# Autodesk Inventor assembly: Assembly-payload-part1
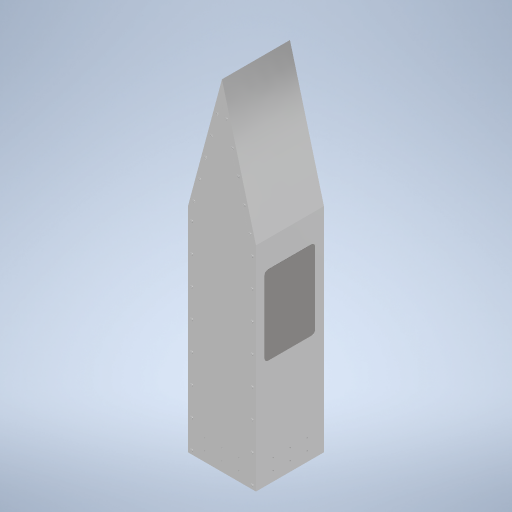
[picture p0: Inventor's stored thumbnail of the model, 512x512]
Saved by Autodesk Inventor 2023 (Build 270158000, 158)
## iProperties
Created: 2023-04-06
Part Number: Assembly-payload-part1
Document SubType Name: Assembly
Designer: ASARe-DAQ-PC
Mass: 73218.4 g
Surface Area: 104206 cm^2
Volume: 27117.9 cm^3
Density: 2.7 g/cm^3
Author: ASARe-DAQ-PC
## Documents named in this file (17)
- C:\Users\310611102\Documents\Inventor\SSR\avionics_2023ver\Payload\Assembly-payload-part1.iam
- C:\Users\310611102\Documents\Inventor\SSR\avionics_2023ver\Payload\Model Shell_part1_up_plate.ipt
- C:\Users\310611102\Documents\Inventor\SSR\avionics_2023ver\Payload\Model Shell_part1_bottom_plate.ipt
- C:\Users\310611102\Documents\Inventor\SSR\avionics_2023ver\Payload\Model Shell_part1_side_plate.ipt
- C:\Users\310611102\Documents\Inventor\SSR\avionics_2023ver\Payload\Model Shell_part1_tip_plate.ipt
- C:\Users\310611102\Documents\Inventor\SSR\avionics_2023ver\Payload\back_board.ipt
- C:\Users\310611102\Documents\Inventor\SSR\avionics_2023ver\Payload\waterproof_door_on_back_board.ipt
- C:\Users\310611102\Documents\Inventor\SSR\avionics_2023ver\Payload\Screw M4 Hex Flat Head 14mm.ipt
- C:\Users\310611102\Documents\Inventor\SSR\avionics_2023ver\Payload\Screw M3 Hex 12mm.ipt
- C:\Users\310611102\Documents\Inventor\SSR\avionics_2023ver\Payload\Screw M4 Hex Flat Head 10mm.ipt
- C:\Users\310611102\Documents\Inventor\SSR\avionics_2023ver\Payload\Screw M3 Hex 8mm.ipt
- C:\Users\310611102\Documents\Inventor\SSR\avionics_2023ver\Payload\Model Shell_part1_side_plate_no_hole.ipt
- C:\Users\310611102\Documents\Inventor\SSR\avionics_2023ver\Payload\Tip_support_1.ipt
- C:\Users\310611102\Documents\Inventor\SSR\avionics_2023ver\Payload\Mirror_shell3.ipt
- C:\Users\310611102\Documents\Inventor\SSR\avionics_2023ver\Payload\acrylic_for_PSI.ipt
- C:\Users\310611102\Documents\Inventor\SSR\avionics_2023ver\Payload\FSI Plate.ipt
- C:\Users\310611102\Documents\Inventor\SSR\avionics_2023ver\Payload\Model Shell - access panel L.ipt
## Components (81 placed, 16 different names)
1. Model Shell_part1_up_plate:1 — Flush:2, Flush:3, Mate:3, Mate:4, Mate:7, Insert:44, Insert:46, Insert:48, Insert:50, Insert:52, Insert:54, Insert:56, Insert:58, Insert:76, Insert:77, Insert:80, Insert:82, Insert:84, Insert:86, Insert:88, Insert:90, Mate:17, Insert:96, Mate:20, Flush:7, Flush:8, Mate:21, Mate:22, Mate:23
2. Model Shell_part1_bottom_plate:1 — Flush:3, Mate:5, Mate:6, Insert:43, Insert:45, Insert:47, Insert:49, Insert:51, Insert:53, Insert:55, Insert:57, Insert:75, Insert:78, Insert:79, Insert:81, Insert:83, Insert:85, Insert:87, Insert:89, Flush:6, Mate:18, Insert:95
3. Model Shell_part1_side_plate:2 — Flush:2, Mate:3, Mate:4, Mate:5, Mate:6, Flush:4, Mate:9, Flush:5, Insert:1, Insert:2, Insert:91, Insert:94, Mate:24, Insert:101, Insert:102
4. Model Shell_part1_tip_plate:1 — Mate:9, Flush:5, Mate:10, Insert:4, Insert:5, Insert:59, Insert:61, Insert:63, Insert:66, Insert:68, Insert:69, Insert:71, Insert:74
5. Model Shell_part1_tip_plate:2 — Mate:7, Flush:4, Mate:10, Insert:3, Insert:6, Insert:60, Insert:62, Insert:64, Insert:65, Insert:67, Insert:70, Insert:72, Insert:73
6. back_board:1 — Insert:1, Insert:2, Mate:14, Mate:15, Mate:16
7. waterproof_door_on_back_board:1 — Mate:14, Mate:15, Mate:16, Insert:31, Insert:32, Insert:33, Insert:34, Insert:35, Insert:36, Insert:37, Insert:38, Insert:39, Insert:40, Insert:41, Insert:42
8. Screw M4 Hex Flat Head 14mm:1 — Insert:3
9. Screw M4 Hex Flat Head 14mm:2 — Insert:4
10. Screw M4 Hex Flat Head 14mm:3 — Insert:5
11. Screw M4 Hex Flat Head 14mm:4 — Insert:6
12. Screw M3 Hex 12mm:1 — Insert:34
13. Screw M3 Hex 12mm:2 — Insert:33
14. Screw M3 Hex 12mm:3 — Insert:32
15. Screw M3 Hex 12mm:4 — Insert:31
16. Screw M3 Hex 12mm:5 — Insert:40
17. Screw M3 Hex 12mm:6 — Insert:41
18. Screw M3 Hex 12mm:7 — Insert:35
19. Screw M3 Hex 12mm:8 — Insert:36
20. Screw M3 Hex 12mm:9 — Insert:37
21. Screw M3 Hex 12mm:10 — Insert:42
22. Screw M3 Hex 12mm:11 — Insert:38
23. Screw M3 Hex 12mm:12 — Insert:39
24. Screw M4 Hex Flat Head 10mm:1 — Insert:66
25. Screw M4 Hex Flat Head 10mm:2 — Insert:65
26. Screw M4 Hex Flat Head 10mm:3 — Insert:64
27. Screw M4 Hex Flat Head 10mm:4 — Insert:63
28. Screw M4 Hex Flat Head 10mm:5 — Insert:62
29. Screw M4 Hex Flat Head 10mm:6 — Insert:61
30. Screw M4 Hex Flat Head 10mm:7 — Insert:60
31. Screw M4 Hex Flat Head 10mm:8 — Insert:59
32. Screw M4 Hex Flat Head 10mm:9 — Insert:58
33. Screw M4 Hex Flat Head 10mm:10 — Insert:57
34. Screw M4 Hex Flat Head 10mm:11 — Insert:56
35. Screw M4 Hex Flat Head 10mm:12 — Insert:55
36. Screw M4 Hex Flat Head 10mm:13 — Insert:54
37. Screw M4 Hex Flat Head 10mm:14 — Insert:53
38. Screw M4 Hex Flat Head 10mm:15 — Insert:52
39. Screw M4 Hex Flat Head 10mm:16 — Insert:51
40. Screw M4 Hex Flat Head 10mm:17 — Insert:50
41. Screw M4 Hex Flat Head 10mm:18 — Insert:49
42. Screw M4 Hex Flat Head 10mm:19 — Insert:48
43. Screw M4 Hex Flat Head 10mm:20 — Insert:47
44. Screw M4 Hex Flat Head 10mm:21 — Insert:46
45. Screw M4 Hex Flat Head 10mm:22 — Insert:45
46. Screw M4 Hex Flat Head 10mm:23 — Insert:43
47. Screw M4 Hex Flat Head 10mm:24 — Insert:44
48. Screw M4 Hex Flat Head 10mm:25 — Insert:90
49. Screw M4 Hex Flat Head 10mm:26 — Insert:89
50. Screw M4 Hex Flat Head 10mm:27 — Insert:87
51. Screw M4 Hex Flat Head 10mm:28 — Insert:88
52. Screw M4 Hex Flat Head 10mm:29 — Insert:85
53. Screw M4 Hex Flat Head 10mm:30 — Insert:86
54. Screw M4 Hex Flat Head 10mm:31 — Insert:83
55. Screw M4 Hex Flat Head 10mm:32 — Insert:84
56. Screw M4 Hex Flat Head 10mm:33 — Insert:81
57. Screw M4 Hex Flat Head 10mm:34 — Insert:82
58. Screw M4 Hex Flat Head 10mm:35 — Insert:79
59. Screw M4 Hex Flat Head 10mm:36 — Insert:80
60. Screw M4 Hex Flat Head 10mm:37 — Insert:77
61. Screw M4 Hex Flat Head 10mm:38 — Insert:78
62. Screw M4 Hex Flat Head 10mm:39 — Insert:76
63. Screw M4 Hex Flat Head 10mm:40 — Insert:75
64. Screw M4 Hex Flat Head 10mm:41 — Insert:73
65. Screw M4 Hex Flat Head 10mm:42 — Insert:74
66. Screw M4 Hex Flat Head 10mm:43 — Insert:72
67. Screw M4 Hex Flat Head 10mm:44 — Insert:71
68. Screw M4 Hex Flat Head 10mm:45 — Insert:70
69. Screw M4 Hex Flat Head 10mm:46 — Insert:69
70. Screw M4 Hex Flat Head 10mm:47 — Insert:67
71. Screw M4 Hex Flat Head 10mm:48 — Insert:68
72. Screw M3 Hex 8mm:1 — Insert:99
73. Screw M3 Hex 8mm:2 — Insert:100
74. Screw M3 Hex 8mm:3 — Insert:98
75. Screw M3 Hex 8mm:4 — Insert:97
76. Model Shell_part1_side_plate_no_hole:1 — Flush:6, Mate:17, Mate:18, Mate:19, Insert:92, Insert:93
77. Tip_support_1:1 — Mate:19, Insert:91, Insert:92, Insert:93, Insert:94
78. Mirror_shell3:1 — Insert:95, Insert:96, Insert:97, Insert:98, Insert:99, Insert:100
79. acrylic_for_PSI:1 — Mate:20, Flush:7, Flush:8
80. FSI Plate:1 — Mate:21, Mate:22, Mate:23
81. Model Shell - access panel L:1 — Mate:24, Insert:101, Insert:102
## Relationships (103: Insert 78, Mate 18, Flush 7)
- Flush:2: Model Shell_part1_up_plate:1 ↔ Model Shell_part1_side_plate:2
- Flush:3: Model Shell_part1_up_plate:1 ↔ Model Shell_part1_bottom_plate:1
- Mate:3: Model Shell_part1_up_plate:1 ↔ Model Shell_part1_side_plate:2
- Mate:4: Model Shell_part1_up_plate:1 ↔ Model Shell_part1_side_plate:2
- Mate:5: Model Shell_part1_bottom_plate:1 ↔ Model Shell_part1_side_plate:2
- Mate:6: Model Shell_part1_bottom_plate:1 ↔ Model Shell_part1_side_plate:2
- Mate:7: Model Shell_part1_up_plate:1 ↔ Model Shell_part1_tip_plate:2
- Flush:4: Model Shell_part1_side_plate:2 ↔ Model Shell_part1_tip_plate:2
- Mate:9: Model Shell_part1_side_plate:2 ↔ Model Shell_part1_tip_plate:1
- Flush:5: Model Shell_part1_side_plate:2 ↔ Model Shell_part1_tip_plate:1
- Mate:10: Model Shell_part1_tip_plate:1 ↔ Model Shell_part1_tip_plate:2
- Insert:1: Model Shell_part1_side_plate:2 ↔ back_board:1
- Insert:2: Model Shell_part1_side_plate:2 ↔ back_board:1
- Mate:14: back_board:1 ↔ waterproof_door_on_back_board:1
- Mate:15: back_board:1 ↔ waterproof_door_on_back_board:1
- Mate:16: back_board:1 ↔ waterproof_door_on_back_board:1
- Insert:3: Model Shell_part1_tip_plate:2 ↔ Screw M4 Hex Flat Head 14mm:1
- Insert:4: Model Shell_part1_tip_plate:1 ↔ Screw M4 Hex Flat Head 14mm:2
- Insert:5: Model Shell_part1_tip_plate:1 ↔ Screw M4 Hex Flat Head 14mm:3
- Insert:6: Model Shell_part1_tip_plate:2 ↔ Screw M4 Hex Flat Head 14mm:4
- Insert:31: waterproof_door_on_back_board:1 ↔ Screw M3 Hex 12mm:4
- Insert:32: waterproof_door_on_back_board:1 ↔ Screw M3 Hex 12mm:3
- Insert:33: waterproof_door_on_back_board:1 ↔ Screw M3 Hex 12mm:2
- Insert:34: waterproof_door_on_back_board:1 ↔ Screw M3 Hex 12mm:1
- Insert:35: waterproof_door_on_back_board:1 ↔ Screw M3 Hex 12mm:7
- Insert:36: waterproof_door_on_back_board:1 ↔ Screw M3 Hex 12mm:8
- Insert:37: waterproof_door_on_back_board:1 ↔ Screw M3 Hex 12mm:9
- Insert:38: waterproof_door_on_back_board:1 ↔ Screw M3 Hex 12mm:11
- Insert:39: waterproof_door_on_back_board:1 ↔ Screw M3 Hex 12mm:12
- Insert:40: waterproof_door_on_back_board:1 ↔ Screw M3 Hex 12mm:5
- Insert:41: waterproof_door_on_back_board:1 ↔ Screw M3 Hex 12mm:6
- Insert:42: waterproof_door_on_back_board:1 ↔ Screw M3 Hex 12mm:10
- Insert:43: Model Shell_part1_bottom_plate:1 ↔ Screw M4 Hex Flat Head 10mm:23
- Insert:44: Model Shell_part1_up_plate:1 ↔ Screw M4 Hex Flat Head 10mm:24
- Insert:45: Model Shell_part1_bottom_plate:1 ↔ Screw M4 Hex Flat Head 10mm:22
- Insert:46: Model Shell_part1_up_plate:1 ↔ Screw M4 Hex Flat Head 10mm:21
- Insert:47: Model Shell_part1_bottom_plate:1 ↔ Screw M4 Hex Flat Head 10mm:20
- Insert:48: Model Shell_part1_up_plate:1 ↔ Screw M4 Hex Flat Head 10mm:19
- Insert:49: Model Shell_part1_bottom_plate:1 ↔ Screw M4 Hex Flat Head 10mm:18
- Insert:50: Model Shell_part1_up_plate:1 ↔ Screw M4 Hex Flat Head 10mm:17
- Insert:51: Model Shell_part1_bottom_plate:1 ↔ Screw M4 Hex Flat Head 10mm:16
- Insert:52: Model Shell_part1_up_plate:1 ↔ Screw M4 Hex Flat Head 10mm:15
- Insert:53: Model Shell_part1_bottom_plate:1 ↔ Screw M4 Hex Flat Head 10mm:14
- Insert:54: Model Shell_part1_up_plate:1 ↔ Screw M4 Hex Flat Head 10mm:13
- Insert:55: Model Shell_part1_bottom_plate:1 ↔ Screw M4 Hex Flat Head 10mm:12
- Insert:56: Model Shell_part1_up_plate:1 ↔ Screw M4 Hex Flat Head 10mm:11
- Insert:57: Model Shell_part1_bottom_plate:1 ↔ Screw M4 Hex Flat Head 10mm:10
- Insert:58: Model Shell_part1_up_plate:1 ↔ Screw M4 Hex Flat Head 10mm:9
- Insert:59: Model Shell_part1_tip_plate:1 ↔ Screw M4 Hex Flat Head 10mm:8
- Insert:60: Model Shell_part1_tip_plate:2 ↔ Screw M4 Hex Flat Head 10mm:7
- Insert:61: Model Shell_part1_tip_plate:1 ↔ Screw M4 Hex Flat Head 10mm:6
- Insert:62: Model Shell_part1_tip_plate:2 ↔ Screw M4 Hex Flat Head 10mm:5
- Insert:63: Model Shell_part1_tip_plate:1 ↔ Screw M4 Hex Flat Head 10mm:4
- Insert:64: Model Shell_part1_tip_plate:2 ↔ Screw M4 Hex Flat Head 10mm:3
- Insert:65: Model Shell_part1_tip_plate:2 ↔ Screw M4 Hex Flat Head 10mm:2
- Insert:66: Model Shell_part1_tip_plate:1 ↔ Screw M4 Hex Flat Head 10mm:1
- Insert:67: Model Shell_part1_tip_plate:2 ↔ Screw M4 Hex Flat Head 10mm:47
- Insert:68: Model Shell_part1_tip_plate:1 ↔ Screw M4 Hex Flat Head 10mm:48
- Insert:69: Model Shell_part1_tip_plate:1 ↔ Screw M4 Hex Flat Head 10mm:46
- Insert:70: Model Shell_part1_tip_plate:2 ↔ Screw M4 Hex Flat Head 10mm:45
- Insert:71: Model Shell_part1_tip_plate:1 ↔ Screw M4 Hex Flat Head 10mm:44
- Insert:72: Model Shell_part1_tip_plate:2 ↔ Screw M4 Hex Flat Head 10mm:43
- Insert:73: Model Shell_part1_tip_plate:2 ↔ Screw M4 Hex Flat Head 10mm:41
- Insert:74: Model Shell_part1_tip_plate:1 ↔ Screw M4 Hex Flat Head 10mm:42
- Insert:75: Model Shell_part1_bottom_plate:1 ↔ Screw M4 Hex Flat Head 10mm:40
- Insert:76: Model Shell_part1_up_plate:1 ↔ Screw M4 Hex Flat Head 10mm:39
- Insert:77: Model Shell_part1_up_plate:1 ↔ Screw M4 Hex Flat Head 10mm:37
- Insert:78: Model Shell_part1_bottom_plate:1 ↔ Screw M4 Hex Flat Head 10mm:38
- Insert:79: Model Shell_part1_bottom_plate:1 ↔ Screw M4 Hex Flat Head 10mm:35
- Insert:80: Model Shell_part1_up_plate:1 ↔ Screw M4 Hex Flat Head 10mm:36
- Insert:81: Model Shell_part1_bottom_plate:1 ↔ Screw M4 Hex Flat Head 10mm:33
- Insert:82: Model Shell_part1_up_plate:1 ↔ Screw M4 Hex Flat Head 10mm:34
- Insert:83: Model Shell_part1_bottom_plate:1 ↔ Screw M4 Hex Flat Head 10mm:31
- Insert:84: Model Shell_part1_up_plate:1 ↔ Screw M4 Hex Flat Head 10mm:32
- Insert:85: Model Shell_part1_bottom_plate:1 ↔ Screw M4 Hex Flat Head 10mm:29
- Insert:86: Model Shell_part1_up_plate:1 ↔ Screw M4 Hex Flat Head 10mm:30
- Insert:87: Model Shell_part1_bottom_plate:1 ↔ Screw M4 Hex Flat Head 10mm:27
- Insert:88: Model Shell_part1_up_plate:1 ↔ Screw M4 Hex Flat Head 10mm:28
- Insert:89: Model Shell_part1_bottom_plate:1 ↔ Screw M4 Hex Flat Head 10mm:26
- Insert:90: Model Shell_part1_up_plate:1 ↔ Screw M4 Hex Flat Head 10mm:25
- Flush:6: Model Shell_part1_bottom_plate:1 ↔ Model Shell_part1_side_plate_no_hole:1
- Mate:17: Model Shell_part1_up_plate:1 ↔ Model Shell_part1_side_plate_no_hole:1
- Mate:18: Model Shell_part1_bottom_plate:1 ↔ Model Shell_part1_side_plate_no_hole:1
- Mate:19: Model Shell_part1_side_plate_no_hole:1 ↔ Tip_support_1:1
- Insert:91: Model Shell_part1_side_plate:2 ↔ Tip_support_1:1
- Insert:92: Model Shell_part1_side_plate_no_hole:1 ↔ Tip_support_1:1
- Insert:93: Model Shell_part1_side_plate_no_hole:1 ↔ Tip_support_1:1
- Insert:94: Model Shell_part1_side_plate:2 ↔ Tip_support_1:1
- Insert:95: Model Shell_part1_bottom_plate:1 ↔ Mirror_shell3:1
- Insert:96: Model Shell_part1_up_plate:1 ↔ Mirror_shell3:1
- Insert:97: Screw M3 Hex 8mm:4 ↔ Mirror_shell3:1
- Insert:98: Screw M3 Hex 8mm:3 ↔ Mirror_shell3:1
- Insert:99: Screw M3 Hex 8mm:1 ↔ Mirror_shell3:1
- Insert:100: Screw M3 Hex 8mm:2 ↔ Mirror_shell3:1
- Mate:20: Model Shell_part1_up_plate:1 ↔ acrylic_for_PSI:1
- Flush:7: Model Shell_part1_up_plate:1 ↔ acrylic_for_PSI:1
- Flush:8: Model Shell_part1_up_plate:1 ↔ acrylic_for_PSI:1
- Mate:21: Model Shell_part1_up_plate:1 ↔ FSI Plate:1
- Mate:22: Model Shell_part1_up_plate:1 ↔ FSI Plate:1
- Mate:23: Model Shell_part1_up_plate:1 ↔ FSI Plate:1
- Mate:24: Model Shell_part1_side_plate:2 ↔ Model Shell - access panel L:1
- Insert:101: Model Shell_part1_side_plate:2 ↔ Model Shell - access panel L:1
- Insert:102: Model Shell_part1_side_plate:2 ↔ Model Shell - access panel L:1
